# Autodesk Inventor assembly: odom_pod
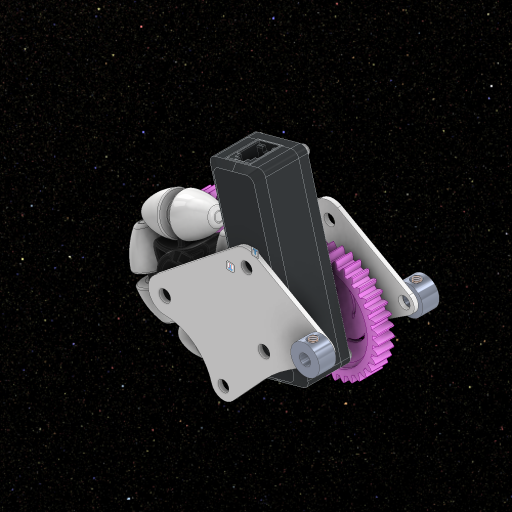
[picture p0: Inventor's stored thumbnail of the model, 512x512]
Saved by Autodesk Inventor 2024 (Build 280153000, 153)
## iProperties
Created: 2024-02-24
Part Number: odom_pod
Document SubType Name: Assembly
Designer: Averey Ku
Author: Averey Ku
## Documents named in this file (6)
- D:\vex_robotics\hardware\cad\vroomba_v0.1\odom_pod.iam
- C:\Users\Averey Ku\Downloads\2” Omni-Directional Wheel (276-9044)\2” Omni-Directional Wheel (276-9044).ipt
- D:\vex_robotics\hardware\cad\vroomba_v0.1\odom_pod.ipt
- D:\vex_robotics\hardware\cad\VEX-CAD-Inventor-1.41\Electronics\Sensors\V5 Rotation Sensor.ipt
- D:\vex_robotics\hardware\cad\VEX-CAD-Inventor-1.41\Motion\Gears\LS 36T Gear.ipt
- D:\vex_robotics\hardware\cad\VEX-CAD-Inventor-1.41\Motion\Shaft LS\Shaft Collar ipts\Shaft Collar No Screw.ipt
## Components (8 placed, 5 different names)
1. 2” Omni-Directional Wheel (276-9044):1 — Insert:5
2. odom_pod:1 — Insert:1, Mate:2, Mate:3, Insert:7, Insert:8
3. V5 Rotation Sensor:1 — Insert:1, Mate:2, Mate:3, Insert:4
4. LS 36T Gear:1 — Insert:4
5. LS 36T Gear:2 — Insert:5, Insert:10
6. odom_pod:2 — Insert:7, Insert:9, Insert:10
7. Shaft Collar No Screw:1 — Insert:9
8. Shaft Collar No Screw:2 — Insert:8
## Relationships (9: Insert 7, Mate 2)
- Insert:1: odom_pod:1 ↔ V5 Rotation Sensor:1
- Mate:2: odom_pod:1 ↔ V5 Rotation Sensor:1
- Mate:3: odom_pod:1 ↔ V5 Rotation Sensor:1
- Insert:4: V5 Rotation Sensor:1 ↔ LS 36T Gear:1
- Insert:5: 2” Omni-Directional Wheel (276-9044):1 ↔ LS 36T Gear:2
- Insert:7 (30.1625 mm): odom_pod:1 ↔ odom_pod:2
- Insert:8: odom_pod:1 ↔ Shaft Collar No Screw:2
- Insert:9: odom_pod:2 ↔ Shaft Collar No Screw:1
- Insert:10: LS 36T Gear:2 ↔ odom_pod:2
